# Autodesk Inventor assembly: Base
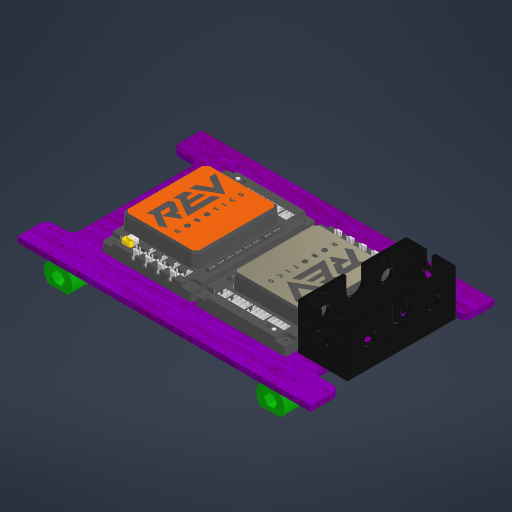
[picture p0: Inventor's stored thumbnail of the model, 512x512]
Saved by Autodesk Inventor 2024.2 (Build 282272000, 272)
## iProperties
Created: 2024-03-15
Part Number: Base
Document SubType Name: Assembly
Designer: Allan Niles
Author: Allan Niles
## Documents named in this file (6)
- C:\Users\alniles07\Documents\Github\8400_2024_CAD\Base.iam
- C:\Users\alniles07\Documents\Github\8400_2024_CAD\Base Plate.ipt
- C:\Users\alniles07\Documents\Github\8400_2024_CAD\Churro Single Mount.ipt
- C:\Users\alniles07\Documents\Github\8400_2024_CAD\Control Hub.ipt
- C:\Users\alniles07\Documents\Github\8400_2024_CAD\Expansion Hub.ipt
- C:\Users\alniles07\Documents\Github\8400_2024_CAD\BatteryMount.ipt
## Components (8 placed, 5 different names)
1. Base Plate:1 — Mate:1, Mate:2, Mate:3, Mate:4, Mate:5, Mate:6, Mate:7, Mate:8, Mate:9, Mate:10, Mate:13
2. Churro Single Mount:1 — Mate:1, Mate:2
3. Churro Single Mount:2 — Mate:3, Mate:4
4. Churro Single Mount:3 — Mate:5, Mate:6
5. Churro Single Mount:4 — Mate:7, Mate:8
6. Control Hub:1
7. Expansion Hub:1 — Mate:9, Mate:10
8. BatteryMount:1 — Mate:13
## Relationships (11: Mate 11)
- Mate:1: Base Plate:1 ↔ Churro Single Mount:1
- Mate:2: Base Plate:1 ↔ Churro Single Mount:1
- Mate:3: Base Plate:1 ↔ Churro Single Mount:2
- Mate:4: Base Plate:1 ↔ Churro Single Mount:2
- Mate:5: Base Plate:1 ↔ Churro Single Mount:3
- Mate:6: Base Plate:1 ↔ Churro Single Mount:3
- Mate:7: Base Plate:1 ↔ Churro Single Mount:4
- Mate:8: Base Plate:1 ↔ Churro Single Mount:4
- Mate:9: Base Plate:1 ↔ Expansion Hub:1
- Mate:10: Base Plate:1 ↔ Expansion Hub:1
- Mate:13: Base Plate:1 ↔ BatteryMount:1
